# Autodesk Inventor assembly: Assemble
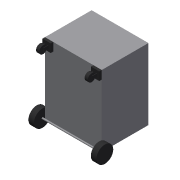
[picture p0: Inventor's stored thumbnail of the model, 180x180]
Saved by Autodesk Inventor 2019 (Build 230136000, 136)
## iProperties
Created: 2019-04-28
Part Number: Assemble
Material: 일반
Document SubType Name: Assembly
Designer: hinmo
Author: hinmo
## Documents named in this file (4)
- C:\Users\hinmo\Documents\Inventor\Projects\2019_CapstoneDesignSimple\Assemble.iam
- C:\Users\hinmo\Documents\Inventor\Projects\2019_CapstoneDesignSimple\Body.ipt
- C:\Users\hinmo\Documents\Inventor\Projects\2019_CapstoneDesignSimple\Wheel.ipt
- C:\Users\hinmo\Documents\Inventor\Projects\2019_CapstoneDesignSimple\Caster.ipt
## Components (5 placed, 3 different names)
1. Body:1 — 메이트:5, 메이트:6, 메이트:7, 메이트:8, 메이트:9, 메이트:10, 메이트:11, 플러쉬:1, 플러쉬:2, 플러쉬:3, 플러쉬:4
2. Wheel:1 — 메이트:4, 메이트:8, 메이트:9
3. Wheel:2 — 메이트:4
4. Caster:1 — 메이트:10, 플러쉬:1, 플러쉬:2
5. Caster:2 — 메이트:11, 플러쉬:3, 플러쉬:4
## Relationships (12: Mate 8, Flush 4)
- 메이트:4 [Mate]: Wheel:1 ↔ Wheel:2
- 메이트:5 [Mate]: Body:1
- 메이트:6 [Mate]: Body:1
- 메이트:7 [Mate]: Body:1
- 메이트:8 [Mate]: Body:1 ↔ Wheel:1
- 메이트:9 [Mate]: Body:1 ↔ Wheel:1
- 메이트:10 [Mate]: Body:1 ↔ Caster:1
- 메이트:11 [Mate]: Body:1 ↔ Caster:2
- 플러쉬:1 [Flush]: Body:1 ↔ Caster:1
- 플러쉬:2 [Flush]: Body:1 ↔ Caster:1
- 플러쉬:3 [Flush]: Body:1 ↔ Caster:2
- 플러쉬:4 [Flush]: Body:1 ↔ Caster:2
